# Autodesk Inventor assembly: Assembly1
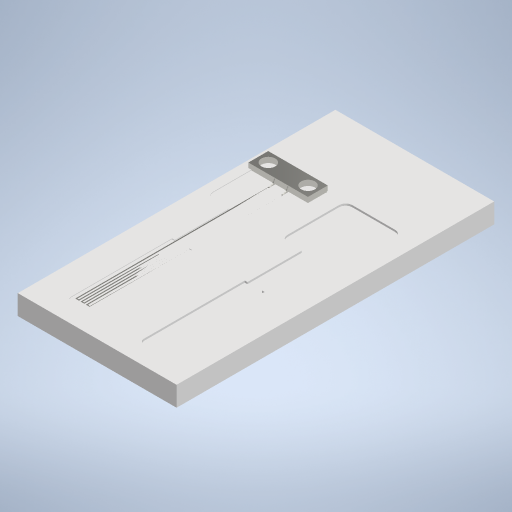
[picture p0: Inventor's stored thumbnail of the model, 512x512]
Saved by Autodesk Inventor 2024.2 (Build 282272000, 272)
## iProperties
Created: 2024-10-29
Part Number: Assembly1
Document SubType Name: Assembly
Designer: Tom
Author: Tom
## Documents named in this file (3)
- C:\Users\Tom\Desktop\UCSF\Preeya UCB\stretchable project\Strain-Sensor-\CAD Files\Sample Holder CNC\plate 1\Assembly1.iam
- C:\Users\Tom\Desktop\UCSF\Preeya UCB\stretchable project\Strain-Sensor-\CAD Files\abs sample design for alignment\strain guage abs 9_17_2024.ipt
- C:\Users\Tom\Desktop\UCSF\Preeya UCB\stretchable project\Strain-Sensor-\CAD Files\Sample Holder CNC\plate 1\0p03_total_thickness.ipt
## Components (2 placed, 2 different names)
1. strain guage abs 9_17_2024:1 — Mate:1, Mate:2
2. 0p03_total_thickness:1 — Mate:1, Mate:2
## Relationships (2: Mate 2)
- Mate:1: strain guage abs 9_17_2024:1 ↔ 0p03_total_thickness:1
- Mate:2: strain guage abs 9_17_2024:1 ↔ 0p03_total_thickness:1
